# Autodesk Inventor assembly: racked
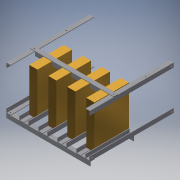
[picture p0: Inventor's stored thumbnail of the model, 180x180]
Saved by Autodesk Inventor 2017 (Build 210142000, 142)
## iProperties
Created: 2018-10-22
Part Number: racked
Document SubType Name: Assembly
Designer: ddeboer
Author: ddeboer
## Documents named in this file (4)
- C:\Users\ddeboer\Desktop\snap_holder\racked_2.iam
- C:\Users\ddeboer\Desktop\snap_holder\bottom.iam
- C:\Users\ddeboer\Desktop\snap_holder\snap.ipt
- C:\Users\ddeboer\Desktop\snap_holder\top_2.iam
## Components (6 placed, 3 different names)
1. bottom:1 [sub-assembly] — Mate:1, Flush:1, Mate:2, Flush:2, Flush:3
2. top_2:1 [sub-assembly] — Flush:2, Flush:3, Mate:3
3. snap:1 — Mate:1, Flush:1, Mate:2, Mate:3
4. snap:2
5. snap:3
6. snap:4
## Component patterns: (4 elements, first: snap:1)
## Relationships (6: Mate 3, Flush 3)
- Mate:1: bottom:1 ↔ snap:1
- Flush:1: bottom:1 ↔ snap:1
- Mate:2: bottom:1 ↔ snap:1
- Flush:2: bottom:1 ↔ top_2:1
- Flush:3: bottom:1 ↔ top_2:1
- Mate:3: top_2:1 ↔ snap:1
